# Autodesk Inventor assembly: ducted fan assembly
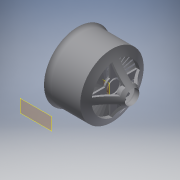
[picture p0: Inventor's stored thumbnail of the model, 180x180]
Saved by Autodesk Inventor 2019 (Build 230136000, 136)
## iProperties
Created: 2020-03-27
Part Number: ducted fan assembly
Document SubType Name: Assembly
Designer: q
Author: q
## Documents named in this file (3)
- C:\Users\q\Desktop\CAD\ducted fan assembly.iam
- C:\Users\q\Desktop\CAD\ducted fan barrel.ipt
- C:\Users\q\Desktop\CAD\fucted fan flades.ipt
## Components (2 placed, 2 different names)
1. ducted fan barrel:1 — Mate:1, Cylindrical:1
2. fucted fan flades:1 — Mate:1, Cylindrical:1
## Relationships (2: Mate 1, CylindricalJoint 1)
- Mate:1: ducted fan barrel:1 ↔ fucted fan flades:1
- Cylindrical:1: ducted fan barrel:1 ↔ fucted fan flades:1
